# Autodesk Inventor assembly: Housing with Camera Cylinder v.02
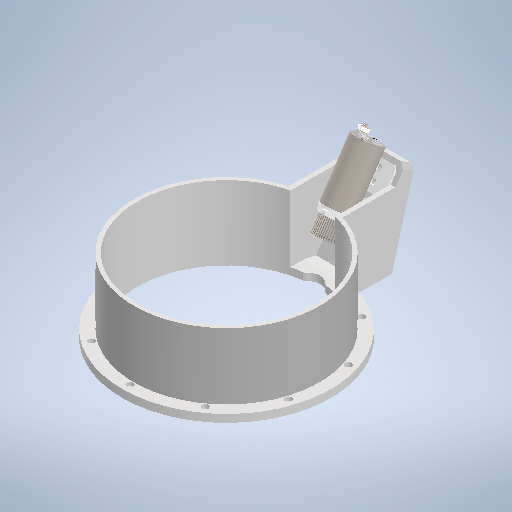
[picture p0: Inventor's stored thumbnail of the model, 512x512]
Saved by Autodesk Inventor 2025.2 (Build 292293000, 293)
## iProperties
Created: 2025-07-30
Part Number: Housing with Camera Cylinder v.02
Document SubType Name: Assembly
Designer: mateo
Author: mateo
## Documents named in this file (3)
- C:\GitHub\In-situ-monitoring-of-powder-bed-fusion-additive-manufacturing\system_development\Mithril\v0.2\Hardware_design\Housing with Camera Cylinder v.02.iam
- C:\GitHub\In-situ-monitoring-of-powder-bed-fusion-additive-manufacturing\system_development\Damascus\v0.2\Hardware\Xi 410 Camera.iam
- C:\GitHub\In-situ-monitoring-of-powder-bed-fusion-additive-manufacturing\system_development\Adamant\v0.2\hardware_development\Cover parts\Cylinder Slidey Bit Housing Camera only v0.2.ipt
## Components (2 placed, 2 different names)
1. Xi 410 Camera:1 [sub-assembly] — Mate:1
2. Cylinder Slidey Bit Housing Camera only v0.2:1 — Mate:1
## Relationships (1: Mate 1)
- Mate:1: Xi 410 Camera:1 ↔ Cylinder Slidey Bit Housing Camera only v0.2:1
